# Autodesk Inventor assembly: Основная часть подъемного механизма первого звена
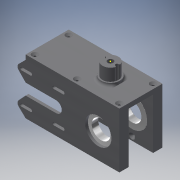
[picture p0: Inventor's stored thumbnail of the model, 180x180]
Saved by Autodesk Inventor 2019.1 (Build 231200000, 200)
## iProperties
Created: 2018-10-15
Part Number: Основная часть подъемного механизма первого звена
Material: Типовые
Document SubType Name: Assembly
Designer: Олег
Author: Олег
## Documents named in this file (5)
- C:\Users\Олег\OneDrive\Общая\NoSpace 2.0\Манипулятор\Основная часть подъемного механизма первого звена.iam
- C:\Users\Олег\OneDrive\Общая\NoSpace 2.0\Манипулятор\Крепление подшипникового блока левая часть.ipt
- C:\Users\Олег\OneDrive\Общая\NoSpace 2.0\Манипулятор\Крепление подшипникового блока правая часть.ipt
- C:\Users\Олег\OneDrive\Общая\NoSpace 2.0\Манипулятор\Основание подъёмного блока первого звена.ipt
- C:\Users\Олег\OneDrive\Общая\NoSpace 2.0\Манипулятор\Подшипник 20х32х7.ipt
## Components (5 placed, 4 different names)
1. Крепление подшипникового блока левая часть:1 — Совмещение:2, Заподлицо:2, Совмещение:4, Заподлицо:5, Заподлицо:6
2. Крепление подшипникового блока правая часть:1 — Совмещение:1, Заподлицо:1, Совмещение:3, Заподлицо:3, Заподлицо:4
3. Основание подъёмного блока первого звена:1 — Совмещение:3, Заподлицо:3, Заподлицо:4, Совмещение:4, Заподлицо:5, Заподлицо:6
4. Подшипник 20х32х7:1 — Совмещение:1, Заподлицо:1
5. Подшипник 20х32х7:2 — Совмещение:2, Заподлицо:2
## Relationships (10: Flush 6, Mate 4)
- Совмещение:1 [Mate]: Крепление подшипникового блока правая часть:1 ↔ Подшипник 20х32х7:1
- Заподлицо:1 [Flush]: Крепление подшипникового блока правая часть:1 ↔ Подшипник 20х32х7:1
- Совмещение:2 [Mate]: Крепление подшипникового блока левая часть:1 ↔ Подшипник 20х32х7:2
- Заподлицо:2 [Flush]: Крепление подшипникового блока левая часть:1 ↔ Подшипник 20х32х7:2
- Совмещение:3 [Mate]: Крепление подшипникового блока правая часть:1 ↔ Основание подъёмного блока первого звена:1
- Заподлицо:3 [Flush]: Крепление подшипникового блока правая часть:1 ↔ Основание подъёмного блока первого звена:1
- Заподлицо:4 [Flush]: Крепление подшипникового блока правая часть:1 ↔ Основание подъёмного блока первого звена:1
- Совмещение:4 [Mate]: Крепление подшипникового блока левая часть:1 ↔ Основание подъёмного блока первого звена:1
- Заподлицо:5 [Flush]: Крепление подшипникового блока левая часть:1 ↔ Основание подъёмного блока первого звена:1
- Заподлицо:6 [Flush]: Крепление подшипникового блока левая часть:1 ↔ Основание подъёмного блока первого звена:1
